# Autodesk Inventor assembly: sestava estonsko
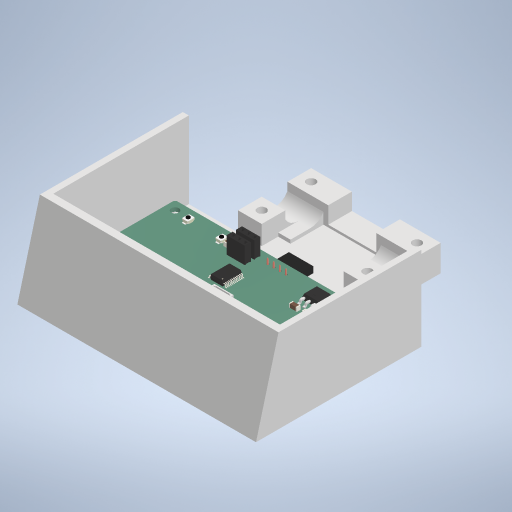
[picture p0: Inventor's stored thumbnail of the model, 512x512]
Saved by Autodesk Inventor 2024 (Build 280153000, 153)
## iProperties
Created: 2023-10-31
Part Number: sestava estonsko
Document SubType Name: Assembly
Designer: Simak
Author: Simak
## Documents named in this file (3)
- C:\Users\Simak\OneDrive\Dokumenty\GitHub\RoboCop\- 3D -\wip\sestava estonsko.iam
- C:\Users\Simak\OneDrive\Dokumenty\GitHub\RoboCop\- 3D -\el._parts\sumec\sumec.ipt
- C:\Users\Simak\OneDrive\Dokumenty\GitHub\RoboCop\- 3D -\wip\tělo estonsko.ipt
## Components (2 placed, 2 different names)
1. tělo estonsko:1 — Proti sobě:1, Vložit:1, Vložit:2
2. sumec:1 — Proti sobě:1, Vložit:1, Vložit:2
## Relationships (3: Insert 2, Mate 1)
- Proti sobě:1 [Mate] (4 mm): tělo estonsko:1 ↔ sumec:1
- Vložit:1 [Insert]: tělo estonsko:1 ↔ sumec:1
- Vložit:2 [Insert]: tělo estonsko:1 ↔ sumec:1
